# Autodesk Inventor assembly: Assembly_Axiovert
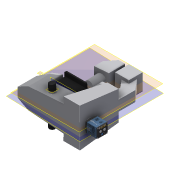
[picture p0: Inventor's stored thumbnail of the model, 180x180]
Saved by Autodesk Inventor 2019.4 (Build 234330000, 330)
## iProperties
Created: 2020-10-09
Part Number: Assembly_Axiovert
Document SubType Name: Assembly
Designer: diederichbenedict
Author: diederichbenedict
## Documents named in this file (5)
- C:\Users\diederichbenedict\Dropbox\Dokumente\Promotion\PROJECTS\STORMoChip\GITHUB\CAD\Nanoscopy-on-the-cheap\Workspace\Assembly_Axiovert.iam
- C:\Users\diederichbenedict\Dropbox\Dokumente\Promotion\PROJECTS\STORMoChip\GITHUB\CAD\Nanoscopy-on-the-cheap\Workspace\00_Axiovert_Base.ipt
- C:\Users\diederichbenedict\Dropbox\Dokumente\Promotion\PROJECTS\STORMoChip\GITHUB\CAD\Nanoscopy-on-the-cheap\Workspace\00_Axiovert_Wheel.ipt
- C:\Users\diederichbenedict\Dropbox\Dokumente\Promotion\PROJECTS\STORMoChip\GITHUB\CAD\Nanoscopy-on-the-cheap\Workspace\00_Axiovert_focusblock.ipt
- C:\Users\diederichbenedict\Dropbox\Dokumente\Promotion\PROJECTS\STORMoChip\GITHUB\CAD\Nanoscopy-on-the-cheap\Workspace\00_PCO_edge-det.ipt
## Components (5 placed, 4 different names)
1. 00_Axiovert_Base:1 — Flush:1, Flush:2, Insert:1, Flush:3, Flush:4, Insert:2
2. 00_Axiovert_Wheel:1 — Flush:1, Flush:2
3. 00_Axiovert_Wheel:2 — Insert:1
4. 00_Axiovert_focusblock:1 — Flush:3, Flush:4
5. 00_PCO_edge-det:1 — Insert:2
## Relationships (6: Flush 4, Insert 2)
- Flush:1: 00_Axiovert_Base:1 ↔ 00_Axiovert_Wheel:1
- Flush:2: 00_Axiovert_Base:1 ↔ 00_Axiovert_Wheel:1
- Insert:1: 00_Axiovert_Base:1 ↔ 00_Axiovert_Wheel:2
- Flush:3: 00_Axiovert_Base:1 ↔ 00_Axiovert_focusblock:1
- Flush:4: 00_Axiovert_Base:1 ↔ 00_Axiovert_focusblock:1
- Insert:2: 00_Axiovert_Base:1 ↔ 00_PCO_edge-det:1
